# Autodesk Inventor assembly: Assemblage ensemble
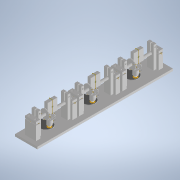
[picture p0: Inventor's stored thumbnail of the model, 180x180]
Saved by Autodesk Inventor 2022 (Build 260153000, 153)
## iProperties
Created: 2021-11-16
Part Number: Assemblage ensemble
Document SubType Name: Assembly
Designer: marti
Author: marti
## iProperties of the stored document MOTOR MODEL 28BYJ-48 5V v4.ipt
Created: 2021-05-29
Part Number: MOTOR MODEL 28BYJ-48 5V v4
Material: Steel
Document SubType Name: Modeling
Designer: marti
Density: 7.85 g/cm^3
Appearance: Par défaut
Sending System: Autodesk Translation Framework v10.9.0.1377
Preprocessor: ST-DEVELOPER v18.1
Title: C:/Users/medua/OneDrive/Escritorio/MOTOR MODEL 28BYJ-48 5V v4.step
## Documents named in this file (12)
- D:\Fac\Projet 2021 Lab Skills\Modelisation\Assemblage ensemble.iam
- D:\Fac\Projet 2021 Lab Skills\Modelisation\plaque_plexi.ipt
- D:\Fac\Projet 2021 Lab Skills\Modelisation\support_paddle.ipt
- D:\Fac\Projet 2021 Lab Skills\Modelisation\pince_fibre.ipt
- D:\Fac\Projet 2021 Lab Skills\Modelisation\support_paddle_MIR.ipt
- D:\Fac\Projet 2021 Lab Skills\Modelisation\pince_fibre_MIR.ipt
- D:\Fac\Projet 2021 Lab Skills\Modelisation\paddle_imp3D.ipt
- **D:\Fac\Projet 2021 Lab Skills\Modelisation\Assemblage ensemble.iam*LocalDocs*xAaaaaycaAaaaaaaaAaaaqrlaUc*MOTOR MODEL 28BYJ-48 5V v4.ipt
- D:\Fac\Projet 2021 Lab Skills\Modelisation\gear_cross_good.ipt
- D:\Fac\Projet 2021 Lab Skills\Modelisation\embout_1b.ipt
- D:\Fac\Projet 2021 Lab Skills\Modelisation\pince_fibre_sup.ipt
- D:\Fac\Projet 2021 Lab Skills\Modelisation\motor-model-28byj-48-5v-1.snapshot.1\MOTOR MODEL 28BYJ-48 5V v4.step
## Components (34 placed, 10 different names)
1. plaque_plexi:1 — Affleurement:6, Placage:15, Angle:5
2. support_paddle:1 — Placage:1, Affleurement:2, Placage:5, Placage:14
3. pince_fibre:1 — Placage:3, Placage:4, Placage:5, Placage:6, Placage:28, Placage:29
4. support_paddle_MIR:1 — Placage:7, Affleurement:3, Placage:9, Placage:13, Placage:18
5. pince_fibre_MIR:1 — Placage:8, Placage:9, Placage:10, Placage:11, Placage:30, Placage:31
6. paddle_imp3D:1 — Placage:13, Placage:14, Placage:16, Placage:17, Angle:5
7. gear_cross_good:1 — Placage:16, Placage:17, Tangente:1, Placage:19, Angle:3
8. gear_cross_good:2 — Affleurement:4, Angle:2, Tangente:2, Placage:20, Placage:21, Placage:22, Affleurement:5
9. embout_1b:1 — Placage:21, Placage:22, Affleurement:5, Placage:24, Placage:27
10. MOTOR MODEL 28BYJ-48 5V v4:1 — Placage:24, Placage:25, Placage:26, Placage:27
11. pince_fibre_sup:1 — Placage:28, Placage:29
12. pince_fibre_sup:4 — Placage:30, Placage:31
13. support_paddle:3
14. pince_fibre:2
15. support_paddle_MIR:2
16. pince_fibre_MIR:2
17. paddle_imp3D:2
18. gear_cross_good:3
19. gear_cross_good:5
20. embout_1b:2
21. MOTOR MODEL 28BYJ-48 5V v4:2
22. pince_fibre_sup:2
23. pince_fibre_sup:5
24. support_paddle:4
25. pince_fibre:3
26. support_paddle_MIR:3
27. pince_fibre_MIR:3
28. paddle_imp3D:3
29. gear_cross_good:4
30. gear_cross_good:6
31. embout_1b:3
32. MOTOR MODEL 28BYJ-48 5V v4:3
33. pince_fibre_sup:3
34. pince_fibre_sup:6
## Component patterns: (3 elements, first: support_paddle:1 + pince_fibre:1 + support_paddle_MIR:1 + pince_fibre_MIR:1 + paddle_imp3D:1 + gear_cross_good:1 + gear_cross_good:2 + embout_1b:1 + MOTOR MODEL 28BYJ-48 5V v4:1 + pince_fibre_sup:1 + pince_fibre_sup:4)
## Relationships (42: Mate 29, Flush 6, Angle 5, Tangent 2)
- Placage:1 [Mate]: support_paddle:1
- Affleurement:1 [Flush] (36 mm)
- Affleurement:6 [Flush]: plaque_plexi:1
- Affleurement:2 [Flush]: support_paddle:1
- Placage:3 [Mate]: pince_fibre:1
- Placage:4 [Mate]: pince_fibre:1
- Placage:5 [Mate]: support_paddle:1 ↔ pince_fibre:1
- Placage:6 [Mate]: pince_fibre:1
- Placage:7 [Mate]: support_paddle_MIR:1
- Affleurement:3 [Flush]: support_paddle_MIR:1
- Placage:8 [Mate]: pince_fibre_MIR:1
- Placage:9 [Mate]: support_paddle_MIR:1 ↔ pince_fibre_MIR:1
- Placage:10 [Mate]: pince_fibre_MIR:1
- Placage:11 [Mate]: pince_fibre_MIR:1
- Placage:12 [Mate] (-36 mm)
- Placage:13 [Mate]: support_paddle_MIR:1 ↔ paddle_imp3D:1
- Placage:14 [Mate]: support_paddle:1 ↔ paddle_imp3D:1
- Placage:15 [Mate]: plaque_plexi:1
- Placage:16 [Mate]: paddle_imp3D:1 ↔ gear_cross_good:1
- Placage:17 [Mate]: paddle_imp3D:1 ↔ gear_cross_good:1
- Placage:18 [Mate]: support_paddle_MIR:1
- Angle:1 (0 deg)
- Tangente:1: gear_cross_good:1
- Affleurement:4 [Flush]: gear_cross_good:2
- Angle:2 (90 deg): gear_cross_good:2
- Placage:19 [Mate]: gear_cross_good:1
- Angle:3 (0 deg): gear_cross_good:1
- Tangente:2: gear_cross_good:2
- Placage:20 [Mate]: gear_cross_good:2
- Placage:21 [Mate]: gear_cross_good:2 ↔ embout_1b:1
- Placage:22 [Mate]: gear_cross_good:2 ↔ embout_1b:1
- Affleurement:5 [Flush] (-2.5 mm): gear_cross_good:2 ↔ embout_1b:1
- Placage:24 [Mate]: embout_1b:1 ↔ MOTOR MODEL 28BYJ-48 5V v4:1
- Placage:25 [Mate]: MOTOR MODEL 28BYJ-48 5V v4:1
- Angle:4 (0 deg)
- Placage:26 [Mate]: MOTOR MODEL 28BYJ-48 5V v4:1
- Placage:27 [Mate] (0.5 mm): embout_1b:1 ↔ MOTOR MODEL 28BYJ-48 5V v4:1
- Angle:5 (0 deg): plaque_plexi:1 ↔ paddle_imp3D:1
- Placage:28 [Mate] (2 mm): pince_fibre:1 ↔ pince_fibre_sup:1
- Placage:29 [Mate]: pince_fibre:1 ↔ pince_fibre_sup:1
- Placage:30 [Mate] (2 mm): pince_fibre_MIR:1 ↔ pince_fibre_sup:4
- Placage:31 [Mate]: pince_fibre_MIR:1 ↔ pince_fibre_sup:4
